# Autodesk Inventor assembly: MotorPulley_ASM
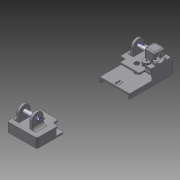
[picture p0: Inventor's stored thumbnail of the model, 180x180]
Saved by Autodesk Inventor 2013 (Build 170138000, 138)
## iProperties
Created: 2013-11-09
Part Number: MotorPulley_ASM
Document SubType Name: Assembly
Designer: JustinIndra
Author: JustinIndra
## Documents named in this file (6)
- C:\Users\JustinIndra\Dropbox\Projects\Mechatronics\Camera Slider\Motorize Kamerar\MotorPulley_ASM.iam
- C:\Users\JustinIndra\Dropbox\Projects\Mechatronics\Camera Slider\Motorize Kamerar\MotorHolder.ipt
- C:\Users\JustinIndra\Dropbox\Projects\Mechatronics\Camera Slider\Motorize Kamerar\PulleyHolder.ipt
- C:\Users\JustinIndra\Dropbox\Projects\Mechatronics\Camera Slider\Motorize Kamerar\PulleyShaft.ipt
- C:\Users\JustinIndra\Dropbox\Projects\Mechatronics\Camera Slider\Motorize Kamerar\MotorMount.ipt
- C:\Users\JustinIndra\Dropbox\Projects\Mechatronics\Camera Slider\Motorize Kamerar\ShaftConverter.ipt
## Components (5 placed, 5 different names)
1. MotorHolder:1 — Flush:1, Flush:2, Mate:3, Mate:4, Mate:5, Mate:6
2. PulleyHolder:1 — Flush:1, Flush:2, Mate:2, Flush:3
3. PulleyShaft:1 — Mate:2, Flush:3
4. MotorMount:1 — Mate:3, Mate:4, Mate:5, Mate:7
5. ShaftConverter:1 — Mate:6, Mate:7
## Relationships (9: Mate 6, Flush 3)
- Flush:1: MotorHolder:1 ↔ PulleyHolder:1
- Flush:2: MotorHolder:1 ↔ PulleyHolder:1
- Mate:2: PulleyHolder:1 ↔ PulleyShaft:1
- Flush:3 (-1 mm): PulleyHolder:1 ↔ PulleyShaft:1
- Mate:3: MotorHolder:1 ↔ MotorMount:1
- Mate:4: MotorHolder:1 ↔ MotorMount:1
- Mate:5: MotorHolder:1 ↔ MotorMount:1
- Mate:6: MotorHolder:1 ↔ ShaftConverter:1
- Mate:7: MotorMount:1 ↔ ShaftConverter:1
